# Autodesk Inventor assembly: ASSEMBLY_Antenna_Case_Top
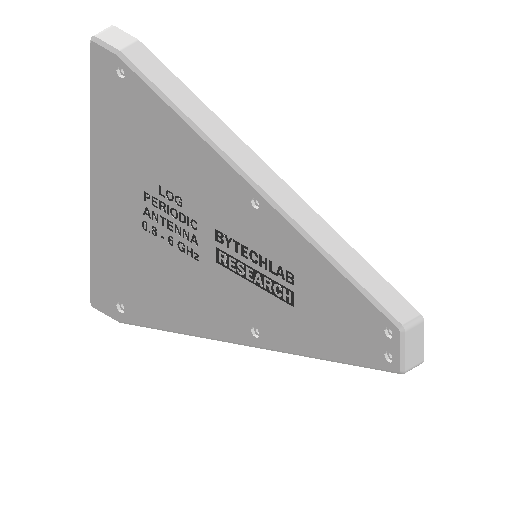
[picture p0: Inventor's stored thumbnail of the model, 512x512]
Saved by Autodesk Inventor 2026.1 (Build 301233000, 233)
## iProperties
Created: 2025-11-20
Part Number: ASSEMBLY_Antenna_Case_Top
Document SubType Name: Assembly
Designer: User
Author: User
## Documents named in this file (3)
- C:\Users\Andrzej\OneDrive\_DRIVE_SYNCH_FILES\RFC - #2 PCB Log Periodic Antenna (0.8-6 GHz)\MCAD\3_WITH_CASE_AND_FEED_COAX_FR4_V1\ASSEMBLY_MAIN_REVA\ASSEMBLY_Antenna_Case_Top.iam
- C:\Users\Andrzej\OneDrive\_DRIVE_SYNCH_FILES\RFC - #2 PCB Log Periodic Antenna (0.8-6 GHz)\MCAD\3_WITH_CASE_AND_FEED_COAX_FR4_V1\ASSEMBLY_MAIN_REVA\3DP_PLA_Antenna_Case_Top.ipt
- C:\Users\Andrzej\OneDrive\_DRIVE_SYNCH_FILES\RFC - #2 PCB Log Periodic Antenna (0.8-6 GHz)\MCAD\3_WITH_CASE_AND_FEED_COAX_FR4_V1\ASSEMBLY_MAIN_REVA\3DP_PLA_Antenna_Case_Top_Logo_and_Name.ipt
## Components (2 placed, 2 different names)
1. 3DP_PLA_Antenna_Case_Top:1 — Mate:1, Mate:2, Mate:3
2. 3DP_PLA_Antenna_Case_Top_Logo_and_Name:1 — Mate:1, Mate:2, Mate:3
## Relationships (3: Mate 3)
- Mate:1: 3DP_PLA_Antenna_Case_Top:1 ↔ 3DP_PLA_Antenna_Case_Top_Logo_and_Name:1
- Mate:2: 3DP_PLA_Antenna_Case_Top:1 ↔ 3DP_PLA_Antenna_Case_Top_Logo_and_Name:1
- Mate:3: 3DP_PLA_Antenna_Case_Top:1 ↔ 3DP_PLA_Antenna_Case_Top_Logo_and_Name:1
